# Autodesk Inventor assembly: Rührreaktor
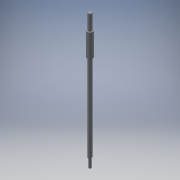
[picture p0: Inventor's stored thumbnail of the model, 180x180]
Saved by Autodesk Inventor 2017 (Build 210142000, 142)
## iProperties
Created: 2019-06-21
Part Number: Rührreaktor
Document SubType Name: Assembly
Designer: Ole Simmering
Author: Ole Simmering
## Documents named in this file (9)
- C:\Users\Ole Simmering\Documents\3d modelling fun\HA5-Rührreaktor\Rührreaktor.iam
- C:\Users\Ole Simmering\Documents\3d modelling fun\HA5-Rührreaktor\Deckelplatte.ipt
- C:\Users\Ole Simmering\Documents\3d modelling fun\HA5-Rührreaktor\Reaktor.ipt
- C:\Users\Ole Simmering\Documents\3d modelling fun\HA5-Rührreaktor\Steckhülse.ipt
- C:\Users\Ole Simmering\Documents\3d modelling fun\HA5-Rührreaktor\Korbbogenboden.ipt
- C:\Users\Ole Simmering\Documents\3d modelling fun\HA5-Rührreaktor\Lagertopf.ipt
- C:\Users\Ole Simmering\Documents\Inventor\Content Center Files\R2017\en-US\DIN 628 SKF(4)\DIN 628 SKF - SKF 7201 BEP.ipt
- C:\Users\Ole Simmering\Documents\3d modelling fun\HA5-Rührreaktor\LagerDeckel.ipt
- C:\Users\Ole Simmering\Documents\3d modelling fun\HA5-Rührreaktor\Achse.ipt
## Components (9 placed, 8 different names)
1. Deckelplatte:1 — Mate:1, Mate:2, Cylindrical:1, Mate:7
2. Reaktor:1 — Mate:1, Mate:2, Mate:3, Mate:4, Mate:5
3. Steckhülse:1 — Insert:3, Mate:11
4. Korbbogenboden:1 — Mate:3, Mate:4, Mate:5
5. Lagertopf:1 — Cylindrical:1, Mate:6, Mate:7, Mate:8, Mate:9, Insert:1
6. DIN 628 SKF - 7..B SKF 7201 BEP:1 — Mate:6, Mate:8, Insert:2
7. DIN 628 SKF - 7..B SKF 7201 BEP:2 — Mate:9, Mate:10
8. LagerDeckel:1 — Insert:1, Mate:10
9. Achse:1 — Insert:2, Insert:3, Mate:11
## Relationships (15: Mate 11, Insert 3, CylindricalJoint 1)
- Mate:1: Deckelplatte:1 ↔ Reaktor:1
- Mate:2: Deckelplatte:1 ↔ Reaktor:1
- Mate:3: Reaktor:1 ↔ Korbbogenboden:1
- Mate:4: Reaktor:1 ↔ Korbbogenboden:1
- Mate:5: Reaktor:1 ↔ Korbbogenboden:1
- Cylindrical:1: Deckelplatte:1 ↔ Lagertopf:1
- Mate:6: Lagertopf:1 ↔ DIN 628 SKF - 7..B SKF 7201 BEP:1
- Mate:7: Deckelplatte:1 ↔ Lagertopf:1
- Mate:8: Lagertopf:1 ↔ DIN 628 SKF - 7..B SKF 7201 BEP:1
- Mate:9: Lagertopf:1 ↔ DIN 628 SKF - 7..B SKF 7201 BEP:2
- Insert:1 (-10 mm): Lagertopf:1 ↔ LagerDeckel:1
- Insert:2: DIN 628 SKF - 7..B SKF 7201 BEP:1 ↔ Achse:1
- Mate:10: DIN 628 SKF - 7..B SKF 7201 BEP:2 ↔ LagerDeckel:1
- Insert:3: Steckhülse:1 ↔ Achse:1
- Mate:11: Steckhülse:1 ↔ Achse:1
